# Autodesk Inventor assembly: MG-IR Sender
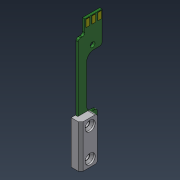
[picture p0: Inventor's stored thumbnail of the model, 180x180]
Saved by Autodesk Inventor 2022.1 (Build 261234020, 234B)
## iProperties
Part Number: MG-IR Sender
Material: Generisch
Document SubType Name: Assembly
Designer: rYan
Mass: 0.541491 g
Surface Area: 12.8728 cm^2
Volume: 0.607715 cm^3
Density: 0.891028 g/cm^3
Author: rYan
## Documents named in this file (4)
- D:\TIGERsGIT\Hardware\mechanik\2020\Inventor\Robot\Electronics\MG-IR Sender.iam
- D:\TIGERsGIT\Hardware\mechanik\2020\Inventor\Robot\Electronics\IR Platine.ipt
- D:\TIGERsGIT\Hardware\mechanik\2020\Inventor\Purchased Parts\IR LED Reverse Gullwing.ipt
- D:\TIGERsGIT\Hardware\mechanik\2020\Inventor\Robot\Dribbler\IR Schutz.ipt
## Components (3 placed, 3 different names)
1. IR Platine:1 — Fluchtend:1, Fluchtend:2, Fluchtend:3, Passend:1, Winkel:1, Passend:2, Einfügen:1, Passend:3
2. IR LED Reverse Gullwing:1 — Passend:1, Winkel:1, Passend:2
3. IR Schutz:1 — Einfügen:1, Passend:3
## Relationships (8: Flush 3, Mate 3, Angle 1, Insert 1)
- Fluchtend:1 [Flush]: IR Platine:1
- Fluchtend:2 [Flush]: IR Platine:1
- Fluchtend:3 [Flush]: IR Platine:1
- Passend:1 [Mate]: IR Platine:1 ↔ IR LED Reverse Gullwing:1
- Winkel:1 [Angle] (0 deg): IR Platine:1 ↔ IR LED Reverse Gullwing:1
- Passend:2 [Mate]: IR Platine:1 ↔ IR LED Reverse Gullwing:1
- Einfügen:1 [Insert]: IR Platine:1 ↔ IR Schutz:1
- Passend:3 [Mate]: IR Platine:1 ↔ IR Schutz:1
